# Autodesk Inventor assembly: Turbina
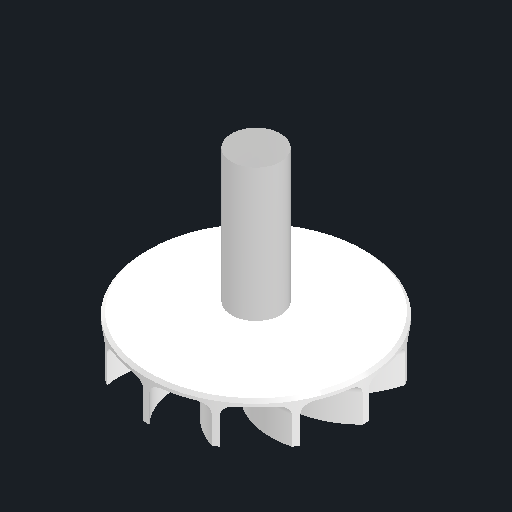
[picture p0: Inventor's stored thumbnail of the model, 512x512]
Saved by Autodesk Inventor 2026.1 (Build 301233020, 233B)
## iProperties
Created: 2026-02-13
Part Number: Turbina
Document SubType Name: Assembly
Designer: celio
Author: celio
## Documents named in this file (3)
- C:\Users\celio\OneDrive\Documentos\Inventor\ZeGuia\Montagem\Turbina\Turbina.iam
- C:\Users\celio\OneDrive\Documentos\Inventor\ZeGuia\Montagem\Turbina\Helice\Helice.ipt
- C:\Users\celio\OneDrive\Documentos\Inventor\ZeGuia\Motores\Coreless\coreless_8523.ipt
## Components (2 placed, 2 different names)
1. Helice:1 — Alinhado:1, Inserir:1
2. coreless_8523:1 — Inserir:1
## Relationships (2: Flush 1, Insert 1)
- Alinhado:1 [Flush]: Helice:1
- Inserir:1 (-4 mm): Helice:1 ↔ coreless_8523:1
